# Autodesk Inventor assembly: BNT 1605-2.6 ZZ+346L C7T(3000)
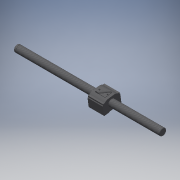
[picture p0: Inventor's stored thumbnail of the model, 180x180]
Saved by Autodesk Inventor 2016 (Build 200138000, 138)
## iProperties
Category: PARTsolutions
Company: THK
Created: 2017-05-16
Part Number: BNT 1605-2.6 ZZ+346L C7T(3000)
Catalog Web Link: www.cadenas.de
Description: Rectangular-Nut Non-Preloaded Type BNT-
Vendor: THK
Document SubType Name: Assembly
Designer: psAdmin
Manufacturer: THK
PSOL_IDENT_0: {$CADENAS_DATA\23d-libs\thk\fed_screw\ball_screw\ball_screw\standard_lead_rbs\bnt_asmtab.prj},258 {V
PSOL_IDENT_1: TYP=3D},{STYP=ASSTAB},{NB=BNT 1605-2.6 ZZ+346L C7T(3000)},{LINA=BNT 1605-2.6 ZZ+346L C7T},{NN=Rectan
PSOL_IDENT_2: gular-Nut Non-Preloaded Type BNT},{DATE=01.12.2014 12:50:12},{GEOMDATE=01.12.2014 12:50:12},{VERSION=
PSOL_IDENT_3: },{LINEID=10},{LINESUBID=-1},{WBVAR=TS,ST,FS,SS,A,PN}  {NB=BNT 1605-2.6 ZZ+346L C7T(3000)},{LINA=BNT
PSOL_IDENT_4: 1605-2.6 ZZ+346L C7T},{KT=DUMMY},{TP=BNT series},{MN=BNT 1605-2.6},{TS=ZZ},{ST=300},{NOTE1=There is
PSOL_IDENT_5: the groove on both ends of the stroke.},{FS=},{INFO1=Infotext},{SS=},{INFO2=Infotext},{OL=346},{NOT
PSOL_IDENT_6: E2=Overall thread lenght is added to the both ends of the stroke 5 mm.},{A=C7},{PN=0},{C7=1500.000},
PSOL_IDENT_7: {C8=1800.000},{C10=1800.000},{FSX='','None','-H1','Type_H1','-H2','Type_H2','-H3','Type_H3','-J1','T
PSOL_IDENT_8: ype_J1','-J2','Type_J2','-J3','Type_J3'},{E3=11},{E4=11},{F1=15},{E1=39},{N1=6},{H1=8},{F2=15},{E2=3
PSOL_IDENT_9: 6},{N2=6},{H2=8},{SD=16},{STX=1675},{EL=1711},{L=36},{FSX1=0},{SSX1=0},{AX1='C7','C7','C8','C8','','
PSOL_IDENT_10: C10'},{PNX=150},{SS1=},{PPATH=bnt/bnt_asmtpl.prj},{INFO1X=fixed_},{INFO2X=supported_}
NN: Rectangular-Nut Non-Preloaded Type BNT
NB: BNT 1605-2.6 ZZ+346L C7T(3000)
NBSYN: $MN. $TS.+$OL.L $A.T$FS.$SS1.($ST.$PN.$SS.)
LINA: BNT 1605-2.6 ZZ+346L C7T
MN: BNT 1605-2.6
TS: ZZ- Brush seals attached on both sides
ST: 300
NOTE1: There is the groove on both ends of the stroke.
INFO1: Infotext
INFO2: Infotext
OL: 346.000
NOTE2: Overall thread lenght is added to the both ends of the stroke 5 mm.
A: C7
PN: 0
SUPPLIER: THK
ARTICLENO: BNT 1605-2.6 ZZ+346L C7T(3000)
BOMINFO: BNT 1605-2.6 ZZ+346L C7T
CREATOR: CADENAS GmbH
Title: BNT 1605-2.6 ZZ+346L C7T
Author: Cadenas PARTsolutions
## Documents named in this file (3)
- C:\Users\M227562\Documents\My Stuff\Ball Screw 1605\BNT 1605-2_6 ZZ+346L C7T(3000).iam
- C:\Users\M227562\Documents\My Stuff\TEST\BNT 1605-2_6300 Shaft.ipt
- C:\Users\M227562\Documents\My Stuff\TEST\BNT 1605-2_6 Nut.ipt
## Components (2 placed, 2 different names)
1. BNT 1605-2_6300 Shaft:1 — Mate:1
2. BNT 1605-2_6 Nut:1 — Mate:1
## Relationships (1: Mate 1)
- Mate:1: BNT 1605-2_6300 Shaft:1 ↔ BNT 1605-2_6 Nut:1
